# Autodesk Inventor assembly: Assembly1
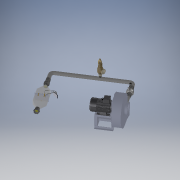
[picture p0: Inventor's stored thumbnail of the model, 180x180]
Saved by Autodesk Inventor 2017 (Build 210142000, 142)
## iProperties
Created: 2017-02-09
Part Number: Assembly1
Document SubType Name: Assembly
Designer: XuZhiqing
Author: XuZhiqing
## Documents named in this file (11)
- C:\Users\XuZhiqing\Desktop\Project01-APS490-CAD-CFD2\CAD-Whole Sys Final\ZSYSTEM\Assembly1.iam
- C:\Users\XuZhiqing\Desktop\Project01-APS490-CAD-CFD2\CAD-Whole Sys Final\safety relief valve\SRV.ipt
- C:\Users\XuZhiqing\Desktop\Project01-APS490-CAD-CFD2\CAD-Whole Sys Final\filter and gauge\filter and gauge\filter and gauge.iam
- C:\Users\XuZhiqing\Desktop\Project01-APS490-CAD-CFD2\CAD-Whole Sys Final\butterfly valve\Butterfly-valve-DIN-11850-male-male-DN50-open.ipt
- C:\Users\XuZhiqing\Desktop\Project01-APS490-CAD-CFD2\CAD-Whole Sys Final\ZSYSTEM\blower.ipt
- C:\Users\XuZhiqing\Desktop\Project01-APS490-CAD-CFD2\CAD-Whole Sys Final\ZSYSTEM\connector1.ipt
- C:\Users\XuZhiqing\Desktop\Project01-APS490-CAD-CFD2\CAD-Whole Sys Final\other\banjo male cam.ipt
- C:\Users\XuZhiqing\Desktop\Project01-APS490-CAD-CFD2\CAD-Whole Sys Final\other\big bend.ipt
- C:\Users\XuZhiqing\Desktop\Project01-APS490-CAD-CFD2\CAD-Whole Sys Final\ZSYSTEM\connector2.ipt
- C:\Users\XuZhiqing\Desktop\Project01-APS490-CAD-CFD2\CAD-Whole Sys Final\ZSYSTEM\Basic Calculator.ipt
- C:\Users\XuZhiqing\Desktop\Project01-APS490-CAD-CFD2\CAD-Whole Sys Final\ZSYSTEM\17032101.ipt
## Components (13 placed, 10 different names)
1. SRV:2 — Mate:17, Mate:18
2. filter and gauge:1 [sub-assembly] — Angle:3, Angle:4, Mate:9, Mate:16, Angle:5, Flush:3
3. Butterfly-valve-DIN-11850-male-male-DN50-open:1 — Angle:1, Mate:1, Mate:8, Mate:13, Mate:15
4. blower:1 — Flush:1, Flush:2, Angle:1, Angle:2, Mate:12
5. connector1:1 — Flush:1, Flush:2, Mate:1, Mate:2, Mate:3, Mate:12
6. banjo male cam:1 — Mate:2, Mate:3, Mate:13
7. connector2:1 — Mate:4, Mate:5, Mate:6, Mate:7, Angle:2, Angle:4, Mate:10
8. banjo male cam:2 — Mate:4, Mate:5, Mate:8, Mate:15
9. banjo male cam:3 — Mate:6, Mate:7, Angle:3, Mate:9, Mate:16
10. big bend:1 — Mate:10, Angle:5, Mate:17, Mate:18
11. Basic Calculator:1 — Flush:3, Mate:19, Mate:20, Mate:21, Mate:22
12. 17032101:1 — Mate:19, Mate:20
13. 17032101:2 — Mate:21, Mate:22
## Relationships (28: Mate 20, Angle 5, Flush 3)
- Flush:1: blower:1 ↔ connector1:1
- Flush:2: blower:1 ↔ connector1:1
- Angle:1 (0 deg): Butterfly-valve-DIN-11850-male-male-DN50-open:1 ↔ blower:1
- Mate:1: Butterfly-valve-DIN-11850-male-male-DN50-open:1 ↔ connector1:1
- Mate:2: connector1:1 ↔ banjo male cam:1
- Mate:3: connector1:1 ↔ banjo male cam:1
- Mate:4: connector2:1 ↔ banjo male cam:2
- Mate:5: connector2:1 ↔ banjo male cam:2
- Mate:6: connector2:1 ↔ banjo male cam:3
- Mate:7: connector2:1 ↔ banjo male cam:3
- Mate:8: Butterfly-valve-DIN-11850-male-male-DN50-open:1 ↔ banjo male cam:2
- Angle:2 (0 deg): blower:1 ↔ connector2:1
- Angle:3 (0 deg): filter and gauge:1 ↔ banjo male cam:3
- Angle:4 (180 deg): filter and gauge:1 ↔ connector2:1
- Mate:9: filter and gauge:1 ↔ banjo male cam:3
- Mate:10: connector2:1 ↔ big bend:1
- Mate:12: blower:1 ↔ connector1:1
- Mate:13: Butterfly-valve-DIN-11850-male-male-DN50-open:1 ↔ banjo male cam:1
- Mate:15: Butterfly-valve-DIN-11850-male-male-DN50-open:1 ↔ banjo male cam:2
- Mate:16: filter and gauge:1 ↔ banjo male cam:3
- Angle:5 (0 deg): filter and gauge:1 ↔ big bend:1
- Mate:17: SRV:2 ↔ big bend:1
- Mate:18: SRV:2 ↔ big bend:1
- Flush:3: filter and gauge:1 ↔ Basic Calculator:1
- Mate:19: Basic Calculator:1 ↔ 17032101:1
- Mate:20: Basic Calculator:1 ↔ 17032101:1
- Mate:21: Basic Calculator:1 ↔ 17032101:2
- Mate:22: Basic Calculator:1 ↔ 17032101:2
